(part 1 of 2)
# Autodesk Inventor assembly: 15InVEX
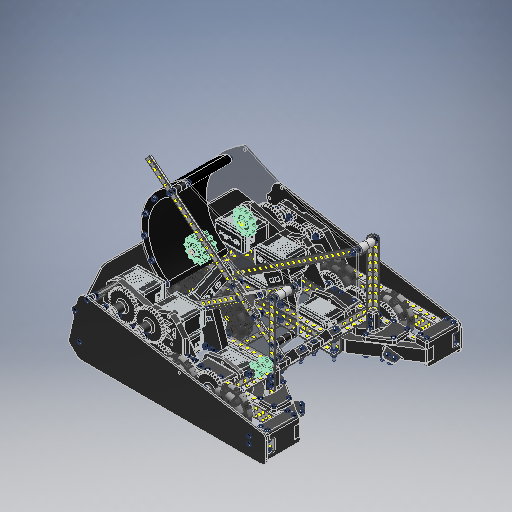
[picture p0: Inventor's stored thumbnail of the model, 512x512]
Saved by Autodesk Inventor 2026.1 (Build 301233000, 233)
## iProperties
Created: 2025-09-07
Part Number: 15InVEX
Document SubType Name: Assembly
Designer: Teddy
Mass: 633.16 g
Surface Area: 4744.79 cm^2
Volume: 520.993 cm^3
Density: 1.2153 g/cm^3
Author: Teddy
## Documents named in this file (80)
- C:\Users\Teddy\Desktop\VexCAD\15InVEX\15InVEX.iam
- C:\Users\Teddy\Desktop\VexCAD\VEX-CAD-Inventor\Structure\C Channel\Aluminum 1x2x1\Alu C 1x2x1x29.ipt
- C:\Users\Teddy\Desktop\VexCAD\VEX-CAD-Inventor\Structure\C Channel\Aluminum 1x3x1\Alu C 1x3x1x29.ipt
- C:\Users\Teddy\Desktop\VexCAD\VEX-CAD-Inventor\Motion\Wheels\Omni Wheel.iam
- C:\Users\Teddy\Desktop\VexCAD\VEX-CAD-Inventor\Structure\Hardware\Screw Steel - Star\SScrew Star Smooth 2.000.ipt
- C:\Users\Teddy\Desktop\VexCAD\VEX-CAD-Inventor\Structure\Hardware\Screw Steel - Star.ipt
- C:\Users\Teddy\Desktop\VexCAD\15InVEX\DriveGear1.ipt
- C:\Users\Teddy\Desktop\VexCAD\VEX-CAD-Inventor\Structure\Hardware\Nut Thin Nylock.ipt
- C:\Users\Teddy\Desktop\VexCAD\VEX-CAD-Inventor\Motion\Insert Circle.ipt
- C:\Users\Teddy\Desktop\VexCAD\15InVEX\DriveGear2.ipt
- C:\Users\Teddy\Desktop\VexCAD\VEX-CAD-Inventor\Motion\Spacers\Spacer Nylon .500 OD.ipt
- C:\Users\Teddy\Desktop\VexCAD\VEX-CAD-Inventor\Motion\Wheels\Omni Wheel\2.75 Omni AS, No Insert.iam
- C:\Users\Teddy\Desktop\VexCAD\VEX-CAD-Inventor\Motion\Insert Square.ipt
- C:\Users\Teddy\Desktop\VexCAD\VEX-CAD-Inventor\Motion\Spacers\Spacer Nylon .500 OD\NSpacer Black .500 OD x .125.ipt
- C:\Users\Teddy\Desktop\VexCAD\VEX-CAD-Inventor\Motion\Spacers\Washer Teflon\TWasher .375 OD x .06250.ipt
- C:\Users\Teddy\Desktop\VexCAD\VEX-CAD-Inventor\Motion\Spacers\Washer Teflon.ipt
- C:\Users\Teddy\Desktop\VexCAD\VEX-CAD-Inventor\Structure\Hardware\Screw Steel - Star\SScrew Star Smooth .250.ipt
- C:\Users\Teddy\Desktop\VexCAD\VEX-CAD-Inventor\Structure\Hardware\Nut Nylock.ipt
- C:\Users\Teddy\Desktop\VexCAD\VEX-CAD-Inventor\Motion\Spacers\Washer Teflon\TWasher .500 OD x .04000.ipt
- C:\Users\Teddy\Desktop\VexCAD\VEX-CAD-Inventor\Motion\Shaft LS\Bearing Flat.ipt
- C:\Users\Teddy\Desktop\VexCAD\VEX-CAD-Inventor\Structure\Hardware\Screw Steel - Star\SScrew Star Smooth .500.ipt
- C:\Users\Teddy\Desktop\VexCAD\VEX-CAD-Inventor\Motion\Spacers\Spacer Nylon .375 OD\NSpacer .375 OD x .250.ipt
- C:\Users\Teddy\Desktop\VexCAD\VEX-CAD-Inventor\Motion\Spacers\Spacer Nylon .375 OD.ipt
- C:\Users\Teddy\Desktop\VexCAD\VEX-CAD-Inventor\Motion\Spacers\Washer Teflon\TWasher .375 OD x .03125.ipt
- C:\Users\Teddy\Desktop\VexCAD\VEX-CAD-Inventor\Structure\Hardware\Screw Steel - Star\SScrew Star Smooth 1.000.ipt
- C:\Users\Teddy\Desktop\VexCAD\15InVEX\CapOriginal.ipt
- C:\Users\Teddy\Desktop\VexCAD\VEX-CAD-Inventor\Structure\Hardware\Screw Steel - Star\SScrew Star Smooth 1.500.ipt
- C:\Users\Teddy\Desktop\VexCAD\VEX-CAD-Inventor\Motion\Shaft LS\Shaft LS.ipt
- C:\Users\Teddy\Desktop\VexCAD\15InVEX\3rdAnd4thGearMount.ipt
- C:\Users\Teddy\Desktop\VexCAD\15InVEX\CombinedMotorMount.ipt
- C:\Users\Teddy\Desktop\VexCAD\VEX-CAD-Inventor\Structure\Hardware\Screw Steel - Star\SScrew Star Smooth .875.ipt
- C:\Users\Teddy\Desktop\VexCAD\VEX-CAD-Inventor\Structure\Hardware\Screw Steel - Star\SScrew Star Smooth 1.750.ipt
- C:\Users\Teddy\Desktop\VexCAD\VEX-CAD-Inventor\Motion\Shaft LS\Shaft LS\Shaft LS 3.5.ipt
- C:\Users\Teddy\Desktop\VexCAD\15InVEX\CombinedMotorMount_MIR.ipt
- C:\Users\Teddy\Desktop\VexCAD\15InVEX\3rdAnd4thGearMount_MIR.ipt
- C:\Users\Teddy\Desktop\VexCAD\15FEBOY\Clamp.ipt
- C:\Users\Teddy\Desktop\VexCAD\VEX-CAD-Inventor\Electronics\V5 Motor No Cap.ipt
- C:\Users\Teddy\Desktop\VexCAD\VEX-CAD-Inventor\Structure\Angle\Aluminum 1x1\Alu Angle 1x1x21.ipt
- C:\Users\Teddy\Desktop\VexCAD\VEX-CAD-Inventor\Structure\C Channel\Aluminum 1x2x1\Alu C 1x2x1x21.ipt
- C:\Users\Teddy\Desktop\VexCAD\VEX-CAD-Inventor\Motion\Spacers\Washer Steel\SWasher .375 OD x .031250.ipt
- C:\Users\Teddy\Desktop\VexCAD\VEX-CAD-Inventor\Motion\Spacers\Washer Steel.ipt
- C:\Users\Teddy\Desktop\VexCAD\VEX-CAD-Inventor\Structure\Hardware\Screw Steel - Star\SScrew Star Smooth .750.ipt
- C:\Users\Teddy\Desktop\VexCAD\15InVEX\Funnel.ipt
- C:\Users\Teddy\Desktop\VexCAD\15InVEX\HardStop.ipt
- C:\Users\Teddy\Desktop\VexCAD\15InVEX\Funnel_MIR.ipt
- C:\Users\Teddy\Desktop\VexCAD\15InVEX\PolyRamp1.ipt
- C:\Users\Teddy\Desktop\VexCAD\15InVEX\Ramp Support.ipt
- C:\Users\Teddy\Desktop\VexCAD\VEX-CAD-Inventor\Structure\Angle\Aluminum 1x1\Alu Angle 1x1x25.ipt
- C:\Users\Teddy\Desktop\VexCAD\15InVEX\AngleSupport.ipt
- C:\Users\Teddy\Desktop\VexCAD\VEX-CAD-Inventor\Structure\Hardware\Screw Steel - Star\SScrew Star Smooth .625.ipt
- C:\Users\Teddy\Desktop\VexCAD\15InVEX\AngleSupport_MIR.ipt
- C:\Users\Teddy\Desktop\VexCAD\VEX-CAD-Inventor\Structure\Angle\Aluminum 1x1\Alu Angle 1x1x15.ipt
- C:\Users\Teddy\Desktop\VexCAD\15InVEX\IntakeSupport.ipt
- C:\Users\Teddy\Desktop\VexCAD\VEX-CAD-Inventor\Motion\Spacers\Spacer Nylon .500 OD\NSpacer White .500 OD x .500.ipt
- C:\Users\Teddy\Desktop\VexCAD\VEX-CAD-Inventor\Motion\Spacers\Spacer Nylon .375 OD\NSpacer .375 OD x .500.ipt
- C:\Users\Teddy\Desktop\VexCAD\VEX-CAD-Inventor\Motion\Spacers\Spacer Nylon .375 OD\NSpacer .375 OD x .375.ipt
- C:\Users\Teddy\Desktop\VexCAD\VEX-CAD-Inventor\Structure\C Channel\Aluminum 1x2x1\Alu C 1x2x1x27.ipt
- C:\Users\Teddy\Desktop\VexCAD\15InVEX\IntakeSupport_MIR.ipt
- C:\Users\Teddy\Desktop\VexCAD\VEX-CAD-Inventor\Structure\Hardware\Screw Steel - Star\SScrew Star Smooth .375.ipt
- C:\Users\Teddy\Desktop\VexCAD\VEX-CAD-Inventor\Structure\Angle\Aluminum 1x1\Alu Angle 1x1x10.ipt
- C:\Users\Teddy\Desktop\VexCAD\VEX-CAD-Inventor\Motion\Wheels\Flex Wheels\1.625 Flex Wheel\1.625 30A .500.ipt
- C:\Users\Teddy\Desktop\VexCAD\VEX-CAD-Inventor\Motion\Wheels\Flex Wheels\1.625 Flex Wheel.ipt
- C:\Users\Teddy\Desktop\VexCAD\VEX-CAD-Inventor\Structure\Angle\Aluminum 1x1\Alu Angle 1x1x26.ipt
- C:\Users\Teddy\Desktop\VexCAD\15InVEX\TwistySupport.ipt
- C:\Users\Teddy\Desktop\VexCAD\VEX-CAD-Inventor\Motion\Sprockets\9P Sprocket\9P 6T Sprocket, Circle.iam
- C:\Users\Teddy\Desktop\VexCAD\VEX-CAD-Inventor\Motion\Sprockets\9P Sprocket.iam
- C:\Users\Teddy\Desktop\VexCAD\VEX-CAD-Inventor\Motion\Spacers\Spacer Nylon .375 OD\NSpacer .375 OD x .125.ipt
- C:\Users\Teddy\Desktop\VexCAD\VEX-CAD-Inventor\Structure\Hardware\Screw Steel - Star\SScrew Star Smooth 2.500.ipt
- C:\Users\Teddy\Desktop\VexCAD\15InVEX\PolyIntakeSides.ipt
- C:\Users\Teddy\Desktop\VexCAD\VEX-CAD-Inventor\Structure\Standoff\Standoff 4.00.ipt
- C:\Users\Teddy\Desktop\VexCAD\VEX-CAD-Inventor\Structure\Standoff.ipt
- C:\Users\Teddy\Desktop\VexCAD\VEX-CAD-Inventor\Motion\Sprockets\9P Sprocket\9P 12T Sprocket, No Insert.iam
- C:\Users\Teddy\Desktop\VexCAD\VEX-CAD-Inventor\Motion\Shaft HS\HS Spacer\HSpacer .1250.ipt
- C:\Users\Teddy\Desktop\VexCAD\VEX-CAD-Inventor\Motion\Shaft HS\HS Spacer.ipt
- C:\Users\Teddy\Desktop\VexCAD\15InVEX\ChassisPolySides.ipt
- C:\Users\Teddy\Desktop\VexCAD\VEX-CAD-Inventor\Structure\Standoff\Standoff 1.50.ipt
- C:\Users\Teddy\Desktop\VexCAD\VEX-CAD-Inventor\Structure\Standoff\Standoff .50.ipt
- C:\Users\Teddy\Desktop\VexCAD\15InVEX\Mesh.ipt
- C:\Users\Teddy\Desktop\VexCAD\15InVEX\BackPoly.ipt
- C:\Users\Teddy\Desktop\VexCAD\VEX-CAD-Inventor\Electronics\Sensors\V5 Rotation Sensor.ipt
## Components (575 placed, 68 different names)
1. SScrew Star Smooth .375:135 — Insert:576
2. SScrew Star Smooth .375:136 — Insert:577
3. Nut Nylock:188 — Insert:579
4. Nut Nylock:189 — Insert:578
5. Alu Angle 1x1x10:1 — Insert:580, Insert:581, Insert:604
6. 1.625 30A .500:1 — Insert:581
7. 1.625 30A .500:2
8. Alu Angle 1x1x26:1 — Insert:582, Flush:20, Insert:584, Insert:585, Insert:586, Insert:587, Insert:598, Insert:599, Insert:606, Insert:607
9. TwistySupport:1 — Flush:18, Flush:19, Flush:20, Insert:583, Insert:584, Insert:585, Insert:588, Insert:589, Insert:590, Insert:593
10. SScrew Star Smooth .750:137 — Insert:586
11. SScrew Star Smooth .750:138 — Insert:587
12. SScrew Star Smooth .750:139 — Insert:588
13. SScrew Star Smooth .750:140 — Insert:589
14. Nut Nylock:190 — Insert:593
15. Nut Nylock:191 — Insert:592
16. Nut Nylock:192 — Insert:591
17. Nut Nylock:193 — Insert:590
18. 9P 6T Sprocket, Circle:1 [sub-assembly] — Insert:595, Insert:597
19. 9P 6T Sprocket, Circle:2 [sub-assembly] — Insert:594, Insert:603
20. NSpacer .375 OD x .125:13 — Insert:594, Insert:597
21. NSpacer .375 OD x .125:15 — Insert:595, Insert:580
22. SScrew Star Smooth 2.500:141 — Insert:598
23. Nut Nylock:194 — Insert:599
24. Nut Nylock:195 — Insert:601, Insert:603
25. Nut Nylock:196 — Insert:600, Insert:602
26. TWasher .500 OD x .04000:21 — Insert:602
27. Nut Nylock:197 — Insert:605
28. TWasher .500 OD x .04000:22 — Insert:604, Insert:605
29. PolyIntakeSides:1 — Flush:21, Flush:22, Insert:560, Insert:592, Insert:591, Insert:610, Insert:618, Insert:620, Insert:621, Insert:622, Insert:623, Insert:624, Insert:625, Insert:626, Insert:645, Insert:657, Insert:658, Insert:659, Insert:660, Insert:661, Insert:662
30. SScrew Star Smooth 1.500:142 — Insert:606
31. Nut Nylock:198 — Insert:607, Insert:608
32. Nut Nylock:199 — Insert:610
33. NSpacer .375 OD x .375:16 — Insert:608, Insert:609
34. NSpacer .375 OD x .375:17 — Insert:609
35. SScrew Star Smooth 2.000:143 — Insert:611
36. Nut Nylock:200 — Insert:612, Insert:613
37. NSpacer .375 OD x .500:18 — Insert:614, Insert:615
38. NSpacer .375 OD x .500:20 — Insert:613, Insert:614
39. NSpacer .375 OD x .250:22 — Insert:615, Insert:616
40. TWasher .500 OD x .04000:23 — Insert:616, Insert:617
41. TWasher .500 OD x .04000:24 — Insert:617
42. Nut Nylock:201 — Insert:618
43. SScrew Star Smooth .375:144 — Insert:619
44. Nut Nylock:202 — Insert:620
45. Standoff 4.00:1 — Insert:631, Insert:638
46. Standoff 4.00:2 — Insert:630, Insert:636
47. Standoff 4.00:3 — Insert:629, Insert:635
48. Standoff 4.00:4 — Insert:628, Insert:634
49. Standoff 4.00:5 — Insert:627, Insert:633
50. Standoff 4.00:6 — Insert:632, Insert:637
51. Nut Thin Nylock:24 — Insert:621, Insert:632
52. Nut Thin Nylock:25 — Insert:622, Insert:631
53. Nut Thin Nylock:26 — Insert:623, Insert:630
54. Nut Thin Nylock:27 — Insert:624, Insert:629
55. Nut Thin Nylock:28 — Insert:625, Insert:628
56. Nut Thin Nylock:29 — Insert:626, Insert:627
57. Nut Thin Nylock:30 — Insert:635, Insert:642
58. Nut Thin Nylock:31 — Insert:636, Insert:641
59. Nut Thin Nylock:32 — Insert:638, Insert:640
60. Nut Thin Nylock:33 — Insert:637, Insert:639
61. Nut Thin Nylock:34 — Insert:633, Insert:644
62. Nut Thin Nylock:35 — Insert:634, Insert:643
63. PolyIntakeSides:2 — Insert:639, Insert:640, Insert:641, Insert:642, Insert:643, Insert:644, Insert:646, Insert:651, Insert:652, Insert:653, Insert:654, Insert:655, Insert:656, Flush:26, Flush:27
64. 9P 12T Sprocket, No Insert:3 [sub-assembly] — Insert:650
65. 9P 12T Sprocket, No Insert:4 [sub-assembly] — Insert:648, Insert:649
66. 9P 12T Sprocket, No Insert:5 [sub-assembly] — Insert:647
67. HSpacer .1250:1 — Insert:645, Insert:648
68. HSpacer .1250:2 — Insert:649, Insert:650
69. HSpacer .1250:3 — Insert:646, Insert:647
70. SScrew Star Smooth .750:145 — Insert:651
71. SScrew Star Smooth .750:146 — Insert:652
72. SScrew Star Smooth .750:147 — Insert:654
73. SScrew Star Smooth .750:148 — Insert:653
74. SScrew Star Smooth .750:149 — Insert:655
75. SScrew Star Smooth .750:150 — Insert:656
76. SScrew Star Smooth .750:151 — Insert:658
77. SScrew Star Smooth .750:152 — Insert:657
78. SScrew Star Smooth .750:153 — Insert:659
79. SScrew Star Smooth .750:154 — Insert:662
80. SScrew Star Smooth .750:155 — Insert:661
81. SScrew Star Smooth .750:156 — Insert:660
82. ChassisPolySides:1 — Flush:24, Flush:25, Insert:665, Insert:666, Insert:669, Insert:670, Insert:673, Insert:674, Insert:675, Insert:676, Insert:677, Insert:678
83. Standoff 1.50:7 — Insert:663, Insert:667
84. Standoff 1.50:8 — Insert:664, Insert:668
85. SScrew Star Smooth 1.000:157 — Insert:665
86. SScrew Star Smooth 1.000:158 — Insert:666
87. Nut Nylock:203 — Insert:667
88. Nut Nylock:204 — Insert:668
89. Nut Nylock:205 — Insert:670, Insert:672
90. Nut Nylock:206 — Insert:669, Insert:671
91. NSpacer .375 OD x .125:23 — Insert:671
92. NSpacer .375 OD x .125:24 — Insert:672
93. SScrew Star Smooth 1.000:159 — Insert:674
94. SScrew Star Smooth 1.000:160 — Insert:675
95. SScrew Star Smooth 1.000:161 — Insert:673
96. Standoff .50:9 — Insert:677
97. Standoff .50:10 — Insert:676
98. Standoff .50:11 — Insert:678
99. Nut Nylock:207 — Insert:679
100. Nut Nylock:208 — Insert:681
101. Nut Nylock:209 — Insert:680
102. ChassisPolySides:2 — Insert:682, Insert:683, Insert:684
103. Mesh:1 — Flush:26, Flush:27
104. BackPoly:1 — Flush:28, Flush:29, Insert:685, Insert:686, Insert:687, Insert:688
105. SScrew Star Smooth .500:162 — Insert:685
106. SScrew Star Smooth .500:163 — Insert:686
107. SScrew Star Smooth .500:164 — Insert:687
108. SScrew Star Smooth .500:165 — Insert:688
109. 2.75 Omni AS, No Insert:7 [sub-assembly] — Insert:689, Insert:691
110. 2.75 Omni AS, No Insert:8 [sub-assembly] — Insert:690, Insert:692
111. V5 Rotation Sensor:1 — Insert:691
112. V5 Rotation Sensor:2 — Insert:692
113. Alu Angle 1x1x15:2 — Insert:556, Insert:557, Insert:559, Insert:570, Insert:571, Angle:13, Insert:582, Insert:600, Insert:601, Insert:611, Insert:612
114. Alu Angle 1x1x15:1 — Insert:507, Angle:12, Insert:514, Insert:515, Insert:535, Insert:536
115. Alu Angle 1x1x25:2 — Insert:491, Insert:495, Insert:496, Insert:497, Insert:498, Insert:556, Insert:558, Flush:18, Flush:19, Insert:583, Flush:21, Flush:22, Insert:619
116. Alu Angle 1x1x25:1 — Insert:476, Insert:479, Insert:480, Insert:489, Insert:490, Insert:507, Insert:516, Insert:517
117. Alu C 1x2x1x21:2 — Insert:344, Insert:345, Insert:351, Insert:353, Insert:354, Insert:359, Insert:360, Insert:364, Insert:367, Insert:368, Insert:375, Insert:491, Insert:492, Insert:493, Insert:494, Insert:504, Insert:505, Insert:506, Insert:576, Insert:577, Flush:23, Insert:689
118. Alu C 1x2x1x21:1 — Insert:343, Insert:346, Insert:352, Insert:355, Insert:356, Insert:361, Insert:362, Insert:363, Insert:372, Insert:373, Insert:376, Insert:476, Flush:13, Mate:19, Mate:20, Insert:481, Insert:482, Insert:483, Insert:484, Insert:485
119. Alu C 1x3x1x29:1 — Insert:1, Angle:1, Insert:29, Insert:141, Insert:144, Insert:155, Insert:305, Insert:306, Angle:5, Insert:345, Insert:346, Insert:365, Insert:366, Insert:369, Insert:370, Insert:371, Insert:374, Flush:28, Flush:29, Insert:690
120. Alu Angle 1x1x21:2 — Insert:333, Insert:334, Insert:165, Insert:296, Insert:357, Insert:358
121. Alu Angle 1x1x21:1 — Insert:331, Insert:332, Insert:335, Insert:336, Insert:343, Insert:344, Mate:14, Insert:421, Insert:422, Insert:436, Insert:466, Insert:470
122. V5 Motor No Cap:7 — Mate:17, Insert:474, Angle:10
123. V5 Motor No Cap:8 — Mate:18, Insert:475, Angle:11
124. V5 Motor No Cap:5 — Mate:12, Insert:348, Angle:9
125. V5 Motor No Cap:6 — Mate:11, Insert:347, Angle:8
126. V5 Motor No Cap:3 — Mate:9, Insert:327
127. V5 Motor No Cap:4 — Mate:10, Insert:328
128. V5 Motor No Cap:1 — Mate:7, Insert:325
129. V5 Motor No Cap:2 — Mate:8, Insert:326
130. Nut Nylock:186 — Insert:570
131. Nut Nylock:187 — Insert:571
132. Nut Nylock:183 — Insert:558
133. Nut Nylock:184 — Insert:559, Insert:561
134. Nut Nylock:185 — Insert:560
135. Nut Nylock:181 — Insert:535
136. Nut Nylock:182 — Insert:536
137. Nut Nylock:177 — Insert:525
138. Nut Nylock:178 — Insert:526
139. Nut Nylock:179 — Insert:527
140. Nut Nylock:180 — Insert:528
141. Nut Nylock:174 — Insert:517, Insert:518
142. Nut Nylock:175 — Insert:516
143. Nut Nylock:176 — Insert:515
144. Nut Nylock:169 — Insert:501
145. Nut Nylock:170 — Insert:502
146. Nut Nylock:171 — Insert:503
147. Nut Nylock:172 — Insert:499
148. Nut Nylock:173 — Insert:500
149. Nut Nylock:164 — Insert:477
150. Nut Nylock:165 — Insert:478
151. Nut Nylock:166 — Insert:486
152. Nut Nylock:167 — Insert:488
153. Nut Nylock:168 — Insert:487
154. Nut Nylock:161 — Insert:460
155. Nut Nylock:162 — Insert:470
156. Nut Nylock:163 — Insert:471
157. Nut Nylock:143 — Insert:436
158. Nut Nylock:142 — Insert:430
159. Nut Nylock:137 — Insert:417
160. Nut Nylock:138 — Insert:419
161. Nut Nylock:139 — Insert:418
162. Nut Nylock:140 — Insert:420
163. Nut Nylock:115 — Insert:367
164. Nut Nylock:116 — Insert:368
165. Nut Nylock:117 — Insert:369
166. Nut Nylock:118 — Insert:372
167. Nut Nylock:119 — Insert:370
168. Nut Nylock:120 — Insert:371
169. Nut Nylock:121 — Insert:373
170. Nut Nylock:122 — Insert:374
171. Nut Nylock:109 — Insert:361
172. Nut Nylock:110 — Insert:360
173. Nut Nylock:111 — Insert:363
174. Nut Nylock:112 — Insert:362
175. Nut Nylock:113 — Insert:364
176. Nut Nylock:114 — Insert:359
177. Nut Nylock:103 — Insert:351
178. Nut Nylock:104 — Insert:352
179. Nut Nylock:105 — Insert:355
180. Nut Nylock:106 — Insert:353
181. Nut Nylock:107 — Insert:354
182. Nut Nylock:108 — Insert:356
183. SScrew Star Smooth 1.500:129 — Insert:564
184. SScrew Star Smooth 1.500:130 — Insert:565
185. SScrew Star Smooth 1.500:131 — Insert:566
186. SScrew Star Smooth 1.500:132 — Insert:567
187. SScrew Star Smooth .750:133 — Insert:568
188. SScrew Star Smooth .750:134 — Insert:569
189. SScrew Star Smooth 2.000:128 — Insert:557
190. SScrew Star Smooth .750:126 — Insert:540
191. SScrew Star Smooth .750:127 — Insert:541
192. SScrew Star Smooth 1.500:122 — Insert:539
193. SScrew Star Smooth 1.500:123
194. SScrew Star Smooth 1.500:124 — Insert:538
195. SScrew Star Smooth 1.500:125
196. SScrew Star Smooth 2.000:121 — Insert:514
197. SScrew Star Smooth .750:118 — Insert:504
198. SScrew Star Smooth .750:119 — Insert:505
199. SScrew Star Smooth .750:120 — Insert:506
200. SScrew Star Smooth .750:111 — Insert:484
201. SScrew Star Smooth .750:112 — Insert:483
202. SScrew Star Smooth .750:113 — Insert:485
203. SScrew Star Smooth .625:114 — Insert:489
204. SScrew Star Smooth .625:115 — Insert:490
205. SScrew Star Smooth 1.750:108 — Insert:467
206. SScrew Star Smooth .875:109 — Insert:468
207. SScrew Star Smooth .875:110 — Insert:469
208. SScrew Star Smooth .750:86 — Insert:428
209. SScrew Star Smooth .750:87 — Insert:429
210. SScrew Star Smooth 2.000:88 — Insert:432
211. SScrew Star Smooth .750:82 — Insert:423
212. SScrew Star Smooth .750:83 — Insert:414
213. SScrew Star Smooth .750:84 — Insert:424
214. SScrew Star Smooth .750:85 — Insert:425
215. SScrew Star Smooth 1.500:72 — Insert:358
216. SScrew Star Smooth 1.500:73 — Insert:357
217. SScrew Star Smooth 2.000:74 — Insert:366
218. SScrew Star Smooth 2.000:75 — Insert:365
219. NSpacer .375 OD x .500:9 — Insert:572, Insert:574
220. NSpacer .375 OD x .500:10 — Insert:573, Insert:575
221. NSpacer .375 OD x .375:11 — Insert:574
222. NSpacer .375 OD x .375:12 — Insert:575
223. NSpacer White .500 OD x .500:18 — Insert:561, Insert:562
224. NSpacer White .500 OD x .500:19 — Insert:562, Insert:563
225. TWasher .500 OD x .04000:20 — Insert:563
226. NSpacer .375 OD x .500:5 — Insert:529, Insert:532
227. NSpacer .375 OD x .500:6 — Insert:530, Insert:531
228. NSpacer .375 OD x .375:7 — Insert:531
229. NSpacer .375 OD x .375:8 — Insert:532
230. NSpacer White .500 OD x .500:16 — Insert:518, Insert:519
231. NSpacer White .500 OD x .500:17 — Insert:519, Insert:520
232. TWasher .500 OD x .04000:19 — Insert:520
233. SScrew Star Smooth .625:116 — Insert:497
234. SScrew Star Smooth .625:117 — Insert:498
235. NSpacer Black .500 OD x .125:14 — Insert:376, Insert:378
236. NSpacer Black .500 OD x .125:15 — Insert:375, Insert:377
237. SWasher .375 OD x .031250:1 — Insert:377
238. SWasher .375 OD x .031250:2 — Insert:378
239. IntakeSupport_MIR:1 — Insert:552, Insert:553, Insert:554, Insert:555, Insert:564, Insert:565, Insert:566, Insert:567, Insert:568, Insert:569
240. HardStop:3 — Insert:542, Insert:543, Insert:544, Insert:545, Insert:546, Insert:547
241. AngleSupport_MIR:1 — Insert:492, Insert:493, Insert:494, Insert:495, Insert:496, Insert:499, Insert:500, Insert:501, Insert:502, Insert:503
242. IntakeSupport:1 — Flush:14, Flush:15, Flush:16, Insert:509, Insert:510, Insert:538, Insert:539, Insert:540, Insert:541
243. AngleSupport:1 — Flush:13, Mate:19, Mate:20, Insert:477, Insert:478, Insert:479, Insert:480, Insert:481, Insert:482, Insert:486, Insert:487, Insert:488
244. Funnel:1 — Mate:13, Mate:14, Mate:16, Insert:419, Insert:420, Insert:413, Insert:543, Insert:552, Insert:553, Insert:578, Insert:579
245. Funnel_MIR:1 — Insert:417, Insert:418, Flush:14, Flush:15, Insert:525, Insert:526, Insert:537
246. Ramp Support:1 — Insert:421, Insert:430, Insert:432, Insert:469
247. Ramp Support:2 — Insert:422, Insert:466, Insert:467, Insert:468, Insert:471
248. PolyRamp1:1 — Insert:413, Insert:414, Insert:423, Insert:424, Insert:425, Insert:428, Insert:429
249. Alu C 1x2x1x27:2 — Insert:1, Insert:10, Insert:11, Angle:1, Insert:17, Insert:24, Insert:45, Insert:59, Insert:63, Insert:64, Insert:87, Mate:1, Angle:2, Insert:91, Insert:92, Insert:93, Insert:94, Insert:95, Insert:96, Insert:101, Insert:102, Insert:109, Insert:110, Insert:111, Insert:112, Insert:113, Insert:114, Insert:123, Insert:124, Insert:156, Insert:157, Insert:160, Insert:161, Insert:162, Insert:163, Insert:164, Angle:4, Insert:331, Insert:334, Insert:340, Insert:341, Insert:342, Mate:13, Insert:554, Insert:555, Insert:572, Insert:573
250. Alu C 1x2x1x29:3 — Insert:29, Insert:32, Insert:33, Insert:34, Insert:35, Insert:36, Insert:48, Insert:49, Insert:85, Insert:86, Flush:2, Flush:3, Flush:4, Insert:145, Insert:146, Insert:147, Insert:148, Insert:149, Insert:150, Insert:151, Insert:152, Insert:168, Insert:169, Mate:16, Insert:456, Insert:457, Insert:458, Insert:459, Insert:460, Insert:461, Insert:473, Insert:542, Angle:13, Flush:24, Flush:25, Insert:679, Insert:680, Insert:681
251. Clamp:4 — Insert:323
252. Clamp:1 — Insert:324
253. CapOriginal:1 — Insert:87, Mate:1, Angle:2, Insert:88, Insert:89, Insert:90, Insert:97, Insert:98, Insert:99, Insert:323, Mate:7, Insert:325
254. CapOriginal:2 — Insert:101, Insert:102, Insert:103, Insert:104, Insert:105, Insert:106, Insert:107, Insert:108, Insert:324, Mate:8, Insert:326
255. CombinedMotorMount:1 — Insert:123, Insert:124, Insert:158, Insert:159, Mate:12, Insert:348, Angle:9, Mate:17, Insert:474, Angle:10, Insert:663, Insert:664
256. 3rdAnd4thGearMount:1 — Flush:2, Flush:3, Flush:4, Insert:119, Insert:127, Insert:128, Insert:129, Insert:130, Insert:137, Insert:138, Insert:139, Insert:140, Insert:170, Insert:171, Insert:472, Insert:473
257. DriveGear1:1 — Insert:12, Insert:20, Insert:57, Insert:58, Rotation:4
258. DriveGear1:2 — Insert:18, Insert:50, Insert:51, Insert:52, Insert:54, Insert:55, Insert:56, Rotation:2, Rotation:3
259. DriveGear2:1 — Insert:21, Insert:25, Insert:39, Tangent:1, Flush:1, Rotation:3, Rotation:4, Rotation:5
260. DriveGear2:2 — Insert:46, Insert:78, Insert:81, Rotation:1, Rotation:2
261. DriveGear1:3 — Insert:65, Insert:66, Insert:67, Insert:69, Insert:70, Insert:71, Rotation:1
262. DriveGear2:3 — Tangent:1, Flush:1, Insert:115, Tangent:2, Flush:6, Insert:125, Insert:154, Rotation:5, Rotation:6
263. DriveGear2:4 — Tangent:2, Flush:6, Insert:119, Insert:120, Insert:126, Insert:153, Rotation:6
264. 2.75 Omni AS, No Insert:1 [sub-assembly] — Insert:20, Insert:26, Insert:72, Insert:73
265. 2.75 Omni AS, No Insert:2 [sub-assembly] — Insert:50, Insert:51, Insert:52, Insert:54, Insert:60, Insert:74, Insert:75
266. 2.75 Omni AS, No Insert:3 [sub-assembly] — Insert:69, Insert:70, Insert:71, Insert:76, Insert:77, Insert:82
267. NSpacer Black .500 OD x .125:1 — Insert:22, Insert:23
268. TWasher .375 OD x .06250:1 — Insert:23, Insert:24
269. TWasher .500 OD x .04000:2 — Insert:31
270. NSpacer .375 OD x .250:1 — Insert:40, Insert:41
271. TWasher .375 OD x .03125:3 — Insert:41
272. TWasher .375 OD x .06250:4 — Insert:44, Insert:45
273. NSpacer Black .500 OD x .125:2 — Insert:44, Insert:47
274. TWasher .500 OD x .04000:5 — Insert:62
275. NSpacer .375 OD x .250:2 — Insert:79, Insert:80
276. TWasher .375 OD x .03125:6 — Insert:80
277. TWasher .500 OD x .04000:7 — Insert:84
278. NSpacer Black .500 OD x .125:3 — Insert:116, Insert:117
279. TWasher .375 OD x .06250:8 — Insert:117
280. NSpacer Black .500 OD x .125:4 — Insert:121, Insert:122
281. TWasher .375 OD x .06250:9 — Insert:122
282. NSpacer Black .500 OD x .125:6 — Insert:131
283. NSpacer Black .500 OD x .125:7 — Insert:132
284. Insert Circle:1 — Insert:12, Insert:13
285. Insert Circle:3 — Insert:18, Insert:19
286. Insert Square:1 — Insert:21, Insert:22
287. Insert Circle:4 — Insert:26, Insert:30
288. Insert Square:2 — Insert:39, Insert:40
289. Insert Square:3 — Insert:46, Insert:47
290. Insert Circle:5 — Insert:60, Insert:61
291. Insert Circle:6 — Insert:65, Insert:68
292. Insert Square:4 — Insert:78, Insert:79
293. Insert Circle:7 — Insert:82, Insert:83
294. Insert Square:5 — Insert:115, Insert:116
295. Insert Square:6 — Insert:120, Insert:121
296. Insert Square:7 — Insert:125, Insert:131
297. Insert Square:8 — Insert:126, Insert:132
298. Bearing Flat:1 — Insert:33, Insert:34, Insert:37, Insert:38, Insert:172
299. Bearing Flat:2 — Insert:48, Insert:49, Insert:166, Insert:167, Insert:330
300. Bearing Flat:3 — Insert:127, Insert:128, Insert:135, Insert:136
301. Bearing Flat:4 — Insert:129, Insert:130, Insert:133, Insert:134
302. Nut Nylock:154 — Insert:457
303. Nut Nylock:155 — Insert:459
304. Nut Nylock:156 — Insert:458
305. Nut Nylock:157 — Insert:456
306. Nut Nylock:158
307. Nut Nylock:159 — Insert:461
308. Nut Nylock:160
309. Nut Nylock:100 — Insert:342
310. Nut Nylock:101 — Insert:341
311. Nut Nylock:102 — Insert:340
312. Nut Thin Nylock:1 — Insert:11, Insert:13
313. Nut Thin Nylock:3 — Insert:17, Insert:19
314. Nut Thin Nylock:4 — Insert:37
315. Nut Thin Nylock:5 — Insert:38
316. Nut Nylock:1 — Insert:30, Insert:31
317. Nut Nylock:2 — Insert:32
318. Nut Nylock:3 — Insert:61, Insert:62
319. Nut Thin Nylock:6 — Insert:64, Insert:68
320. Nut Thin Nylock:7 — Insert:72
321. Nut Thin Nylock:8 — Insert:73
322. Nut Thin Nylock:9 — Insert:74
323. Nut Thin Nylock:10 — Insert:75
324. Nut Thin Nylock:11 — Insert:76
325. Nut Thin Nylock:12 — Insert:77
326. Nut Nylock:4 — Insert:83, Insert:84
327. Nut Nylock:5 — Insert:86
328. Nut Nylock:6 — Insert:85
329. Nut Nylock:7 — Insert:93
330. Nut Nylock:8 — Insert:91
331. Nut Nylock:9 — Insert:92
332. Nut Nylock:10 — Insert:97
333. Nut Nylock:11 — Insert:94
334. Nut Nylock:12 — Insert:95
335. Nut Nylock:13 — Insert:98
336. Nut Nylock:14 — Insert:99
337. Nut Nylock:15 — Insert:96
338. Nut Nylock:16 — Insert:106
339. Nut Nylock:17 — Insert:107
340. Nut Nylock:18 — Insert:108
341. Nut Nylock:19 — Insert:109
342. Nut Nylock:20 — Insert:110
343. Nut Nylock:21 — Insert:111
344. Nut Nylock:22 — Insert:112
345. Nut Nylock:23 — Insert:113
346. Nut Nylock:24 — Insert:114
347. Nut Nylock:25
348. Nut Nylock:26 — Insert:133
349. Nut Nylock:27 — Insert:134
350. Nut Nylock:28 — Insert:135
351. Nut Nylock:29 — Insert:136
352. Nut Nylock:30 — Insert:141
353. Nut Nylock:31
354. Nut Nylock:32 — Insert:472
355. Nut Nylock:33 — Insert:149
356. Nut Nylock:34 — Insert:150
357. Nut Nylock:35 — Insert:151
358. Nut Nylock:36 — Insert:147
359. Nut Nylock:37 — Insert:148
360. Nut Nylock:38 — Insert:152
361. Nut Nylock:39 — Insert:156
362. Nut Nylock:40 — Insert:157
363. Nut Nylock:41 — Insert:160
364. Nut Nylock:42 — Insert:161
365. Nut Nylock:43 — Insert:162
366. Nut Nylock:44 — Insert:163
367. Nut Nylock:45 — Insert:165
368. Nut Nylock:46 — Insert:164
369. Nut Nylock:47 — Insert:166
370. Nut Nylock:48 — Insert:167
371. SScrew Star Smooth 1.750:104 — Insert:547
372. SScrew Star Smooth 1.750:105 — Insert:545
373. SScrew Star Smooth 1.750:106 — Insert:546
374. SScrew Star Smooth 1.750:107 — Insert:544
375. SScrew Star Smooth 1.500:68 — Insert:335
376. SScrew Star Smooth 2.000:1 — Insert:10
377. SScrew Star Smooth .250:2 — Insert:25
378. SScrew Star Smooth .500:3 — Insert:36
379. SScrew Star Smooth .500:4 — Insert:35
380. SScrew Star Smooth 1.000:5 — Insert:55
381. SScrew Star Smooth 1.000:6 — Insert:56
382. SScrew Star Smooth 1.000:7 — Insert:58
383. SScrew Star Smooth 1.000:8 — Insert:57
384. SScrew Star Smooth 2.000:9 — Insert:59
385. SScrew Star Smooth 1.000:12 — Insert:67
386. SScrew Star Smooth 2.000:10 — Insert:63
387. SScrew Star Smooth 1.000:13 — Insert:66
388. SScrew Star Smooth .250:14 — Insert:81
389. SScrew Star Smooth 1.500:15 — Insert:88
390. SScrew Star Smooth 1.500:16 — Insert:89
391. SScrew Star Smooth 1.500:17 — Insert:90
392. SScrew Star Smooth 1.500:18 — Insert:103
393. SScrew Star Smooth 1.500:19 — Insert:104
394. SScrew Star Smooth 1.500:20 — Insert:105
395. SScrew Star Smooth .875:21 — Insert:137
396. SScrew Star Smooth .875:22 — Insert:138
397. SScrew Star Smooth .875:23 — Insert:139
398. SScrew Star Smooth .875:24 — Insert:140
399. SScrew Star Smooth 1.750:25 — Insert:144
400. SScrew Star Smooth 1.750:26 — Insert:145
401. SScrew Star Smooth 1.500:27 — Insert:146
402. SScrew Star Smooth .250:28 — Insert:153
403. SScrew Star Smooth .250:29 — Insert:154
404. SScrew Star Smooth 1.750:30 — Insert:155
405. SScrew Star Smooth 1.500:31 — Insert:158
406. SScrew Star Smooth 1.500:32 — Insert:159
407. SScrew Star Smooth .500:33 — Insert:168
408. SScrew Star Smooth .500:34 — Insert:169
409. Shaft LS 3.5:9 — Insert:330
410. Shaft LS 3.5:2 — Insert:170
411. Shaft LS 3.5:3 — Insert:172
412. Shaft LS 3.5:4 — Insert:171
413. Alu C 1x2x1x27:1 — Insert:173, Insert:174, Insert:175, Insert:177, Insert:194, Insert:204, Insert:208, Insert:209, Insert:229, Angle:3, Insert:233, Insert:234, Insert:235, Insert:237, Insert:238, Insert:241, Insert:243, Insert:244, Insert:251, Insert:252, Insert:253, Insert:254, Insert:255, Insert:256, Insert:260, Insert:261, Insert:288, Insert:289, Insert:292, Insert:293, Insert:294, Insert:295, Insert:297, Insert:305, Angle:4, Insert:308, Insert:332, Insert:333, Insert:337, Insert:338, Insert:339, Flush:16, Insert:509, Insert:510, Insert:527, Insert:528, Insert:529, Insert:530
414. Alu C 1x2x1x29:5 — Insert:182, Insert:185, Insert:186, Insert:187, Insert:188, Insert:189, Insert:190, Insert:227, Insert:228, Mate:4, Mate:5, Mate:6, Insert:280, Insert:281, Insert:282, Insert:283, Insert:284, Insert:285, Insert:286, Insert:287, Insert:300, Insert:301, Insert:306, Angle:5, Insert:307, Insert:442, Insert:443, Insert:444, Insert:445, Insert:446, Insert:447, Angle:12, Insert:682, Insert:683, Insert:684
415. HardStop:2 — Insert:537, Insert:548, Insert:549, Insert:550, Insert:551
416. Clamp:2 — Insert:321, Angle:6
417. Clamp:3 — Insert:322, Angle:7
418. DriveGear1:4 — Insert:176, Insert:202, Insert:203
419. DriveGear1:5 — Insert:196, Insert:197, Insert:198, Insert:199, Insert:200, Insert:201
420. DriveGear2:5 — Insert:191, Flush:7, Tangent:3, Insert:310, Insert:319
421. CapOriginal:3 — Insert:229, Angle:3, Insert:230, Insert:231, Insert:232, Insert:236, Insert:239, Insert:240, Insert:308, Insert:321, Angle:6, Mate:9, Insert:327
422. CapOriginal:4 — Insert:243, Insert:244, Insert:245, Insert:246, Insert:247, Insert:248, Insert:249, Insert:250, Insert:322, Mate:10, Insert:328
423. CombinedMotorMount_MIR:1 — Insert:260, Insert:261, Insert:290, Insert:291, Angle:7, Mate:11, Insert:347, Angle:8, Mate:18, Insert:475, Angle:11
424. 3rdAnd4thGearMount_MIR:1 — Mate:4, Mate:5, Mate:6, Insert:265, Insert:266, Insert:267, Insert:268, Insert:274, Insert:275, Insert:276, Insert:277, Insert:302, Insert:304, Insert:307
425. DriveGear2:6 — Insert:221, Insert:309, Insert:320
426. DriveGear1:6 — Insert:210, Insert:211, Insert:212, Insert:213, Insert:214
427. DriveGear2:7 — Flush:7, Tangent:3, Flush:8, Tangent:4, Insert:262, Insert:311, Insert:318
428. DriveGear2:8 — Flush:8, Tangent:4, Insert:263, Insert:315, Insert:317
429. 2.75 Omni AS, No Insert:6 [sub-assembly] — Insert:212, Insert:213, Insert:214, Insert:219, Insert:220, Insert:224
430. 2.75 Omni AS, No Insert:4 [sub-assembly] — Insert:176, Insert:179, Insert:215, Insert:216
431. 2.75 Omni AS, No Insert:5 [sub-assembly] — Insert:196, Insert:197, Insert:198, Insert:199, Insert:205, Insert:217, Insert:218
432. Bearing Flat:5 — Insert:183, Insert:184, Insert:185, Insert:186, Insert:303
433. Bearing Flat:6 — Insert:187, Insert:188, Insert:298, Insert:299, Insert:329
434. Bearing Flat:7 — Insert:265, Insert:266, Insert:272, Insert:273, Insert:314
435. Bearing Flat:8 — Insert:267, Insert:268, Insert:270, Insert:271
436. NSpacer Black .500 OD x .125:8 — Insert:178, Insert:313
437. TWasher .375 OD x .06250:10 — Insert:177, Insert:178
438. TWasher .500 OD x .04000:11 — Insert:181
439. NSpacer .375 OD x .250:3 — Insert:192, Insert:193
440. TWasher .375 OD x .03125:12 — Insert:193
441. TWasher .375 OD x .06250:13 — Insert:194, Insert:195
442. NSpacer Black .500 OD x .125:9 — Insert:195, Insert:312
443. TWasher .500 OD x .04000:14 — Insert:207
444. NSpacer .375 OD x .250:4 — Insert:222, Insert:223
445. TWasher .375 OD x .03125:15 — Insert:223
446. TWasher .500 OD x .04000:16 — Insert:226
447. NSpacer Black .500 OD x .125:10 — Insert:257
448. TWasher .375 OD x .06250:17 — Insert:257
449. NSpacer Black .500 OD x .125:11 — Insert:259, Insert:316
450. TWasher .375 OD x .06250:18 — Insert:259
451. NSpacer Black .500 OD x .125:12 — Insert:264, Insert:314
452. NSpacer Black .500 OD x .125:13 — Insert:269
453. Nut Nylock:145 — Insert:442
454. Nut Nylock:146 — Insert:443
455. Nut Nylock:147
456. Nut Nylock:148 — Insert:444
457. Nut Nylock:150
458. Nut Nylock:151 — Insert:446
459. Nut Nylock:152 — Insert:445
460. Nut Nylock:153 — Insert:447
461. Nut Nylock:97 — Insert:338
462. Nut Nylock:98 — Insert:337
463. Nut Nylock:99 — Insert:339
464. Nut Thin Nylock:13 — Insert:174
465. Nut Thin Nylock:14 — Insert:175
466. Nut Thin Nylock:15 — Insert:184
467. Nut Thin Nylock:16 — Insert:183
468. Nut Nylock:49 — Insert:180, Insert:181
469. Nut Nylock:50 — Insert:182
470. Nut Nylock:51 — Insert:206, Insert:207
471. Nut Thin Nylock:17 — Insert:209
472. Nut Thin Nylock:18 — Insert:215
473. Nut Thin Nylock:19 — Insert:216
474. Nut Thin Nylock:20 — Insert:217
475. Nut Thin Nylock:21 — Insert:218
476. Nut Thin Nylock:22 — Insert:219
477. Nut Thin Nylock:23 — Insert:220
478. Nut Nylock:52 — Insert:225, Insert:226
479. Nut Nylock:53 — Insert:227
480. Nut Nylock:54 — Insert:228
481. Nut Nylock:55 — Insert:233
482. Nut Nylock:56 — Insert:234
483. Nut Nylock:57 — Insert:235
484. Nut Nylock:58 — Insert:236
485. Nut Nylock:59 — Insert:237
486. Nut Nylock:60 — Insert:238
487. Nut Nylock:61 — Insert:239
488. Nut Nylock:62 — Insert:240
489. Nut Nylock:63 — Insert:241
490. Nut Nylock:64 — Insert:248
491. Nut Nylock:65 — Insert:249
492. Nut Nylock:66 — Insert:250
493. Nut Nylock:67 — Insert:251
494. Nut Nylock:68 — Insert:252
495. Nut Nylock:69 — Insert:253
496. Nut Nylock:70 — Insert:254
497. Nut Nylock:71 — Insert:255
498. Nut Nylock:72 — Insert:256
499. Nut Nylock:73
500. Nut Nylock:74 — Insert:270
501. Nut Nylock:75 — Insert:271
502. Nut Nylock:76 — Insert:272
503. Nut Nylock:77 — Insert:273
504. Nut Nylock:78
505. Nut Nylock:79
506. Nut Nylock:80
507. Nut Nylock:81 — Insert:282
508. Nut Nylock:82 — Insert:283
509. Nut Nylock:83 — Insert:284
510. Nut Nylock:84 — Insert:285
511. Nut Nylock:85 — Insert:286
512. Nut Nylock:86 — Insert:287
513. Nut Nylock:87 — Insert:288
514. Nut Nylock:88 — Insert:289
515. Nut Nylock:89 — Insert:292
516. Nut Nylock:90 — Insert:293
517. Nut Nylock:91 — Insert:294
518. Nut Nylock:92 — Insert:295
519. Nut Nylock:93 — Insert:296
520. Nut Nylock:94 — Insert:297
521. Nut Nylock:95 — Insert:298
522. Nut Nylock:96 — Insert:299
523. SScrew Star Smooth 1.750:100 — Insert:548
524. SScrew Star Smooth 1.750:101 — Insert:549
525. SScrew Star Smooth 1.750:102 — Insert:551
526. SScrew Star Smooth 1.750:103 — Insert:550
527. SScrew Star Smooth 1.500:69 — Insert:336
528. SScrew Star Smooth .250:64 — Insert:319
529. SScrew Star Smooth .250:65 — Insert:317
530. SScrew Star Smooth .250:66 — Insert:318
531. SScrew Star Smooth .250:67 — Insert:320
532. SScrew Star Smooth .875:35 — Insert:274
533. SScrew Star Smooth .875:36 — Insert:275
534. SScrew Star Smooth .875:37 — Insert:276
535. SScrew Star Smooth .875:38 — Insert:277
536. SScrew Star Smooth 1.750:39
537. SScrew Star Smooth 1.750:40 — Insert:280
538. SScrew Star Smooth 1.500:41 — Insert:281
539. SScrew Star Smooth 1.750:42
540. SScrew Star Smooth 1.500:43 — Insert:290
541. SScrew Star Smooth 1.500:44 — Insert:291
542. SScrew Star Smooth .500:45 — Insert:300
543. SScrew Star Smooth 2.000:46 — Insert:173
544. SScrew Star Smooth .500:47 — Insert:189
545. SScrew Star Smooth .500:48 — Insert:190
546. SScrew Star Smooth 1.000:49 — Insert:200
547. SScrew Star Smooth 1.000:50 — Insert:201
548. SScrew Star Smooth 1.000:51 — Insert:202
549. SScrew Star Smooth 1.000:52 — Insert:203
550. SScrew Star Smooth 2.000:53 — Insert:204
551. SScrew Star Smooth 1.000:54 — Insert:210
552. SScrew Star Smooth 2.000:55 — Insert:208
553. SScrew Star Smooth 1.000:56 — Insert:211
554. SScrew Star Smooth 1.500:57 — Insert:230
555. SScrew Star Smooth 1.500:58 — Insert:231
556. SScrew Star Smooth 1.500:59 — Insert:232
557. SScrew Star Smooth 1.500:60 — Insert:245
558. SScrew Star Smooth 1.500:61 — Insert:246
559. SScrew Star Smooth 1.500:62 — Insert:247
560. SScrew Star Smooth .500:63 — Insert:301
561. Shaft LS 3.5:10 — Insert:329
562. Shaft LS 3.5:6 — Insert:302
563. Shaft LS 3.5:7 — Insert:303
564. Shaft LS 3.5:8 — Insert:304
565. Insert Circle:8 — Insert:179, Insert:180
566. Insert Square:9 — Insert:191, Insert:192
567. Insert Circle:9 — Insert:205, Insert:206
568. Insert Square:10 — Insert:221, Insert:222
569. Insert Circle:10 — Insert:224, Insert:225
570. Insert Square:11 — Insert:262, Insert:264
571. Insert Square:12 — Insert:263, Insert:269
572. Insert Square:13 — Insert:309, Insert:312
573. Insert Square:14 — Insert:310, Insert:313
574. Insert Square:15 — Insert:311
575. Insert Square:16 — Insert:315, Insert:316
## Relationships (660: Insert 596, Flush 24, Mate 17, Angle 13, RelateRotation 6, Tangent 4)
- Insert:1: Alu C 1x3x1x29:1 ↔ Alu C 1x2x1x27:2
- Insert:10: Alu C 1x2x1x27:2 ↔ SScrew Star Smooth 2.000:1
- Insert:11: Alu C 1x2x1x27:2 ↔ Nut Thin Nylock:1
- Insert:12: DriveGear1:1 ↔ Insert Circle:1
- Insert:13: Insert Circle:1 ↔ Nut Thin Nylock:1
- Angle:1 (-90 deg): Alu C 1x3x1x29:1 ↔ Alu C 1x2x1x27:2
- Insert:17: Alu C 1x2x1x27:2 ↔ Nut Thin Nylock:3
- Insert:18: DriveGear1:2 ↔ Insert Circle:3
- Insert:19: Insert Circle:3 ↔ Nut Thin Nylock:3
- Insert:20: DriveGear1:1 ↔ 2.75 Omni AS, No Insert:1
- Insert:21: DriveGear2:1 ↔ Insert Square:1
- Insert:22: NSpacer Black .500 OD x .125:1 ↔ Insert Square:1
- Insert:23: NSpacer Black .500 OD x .125:1 ↔ TWasher .375 OD x .06250:1
- Insert:24: Alu C 1x2x1x27:2 ↔ TWasher .375 OD x .06250:1
- Insert:25: DriveGear2:1 ↔ SScrew Star Smooth .250:2
- Insert:26: 2.75 Omni AS, No Insert:1 ↔ Insert Circle:4
- Insert:29: Alu C 1x3x1x29:1 ↔ Alu C 1x2x1x29:3
- Insert:30: Insert Circle:4 ↔ Nut Nylock:1
- Insert:31: TWasher .500 OD x .04000:2 ↔ Nut Nylock:1
- Insert:32: Alu C 1x2x1x29:3 ↔ Nut Nylock:2
- Insert:33: Alu C 1x2x1x29:3 ↔ Bearing Flat:1
- Insert:34: Alu C 1x2x1x29:3 ↔ Bearing Flat:1
- Insert:35: Alu C 1x2x1x29:3 ↔ SScrew Star Smooth .500:4
- Insert:36: Alu C 1x2x1x29:3 ↔ SScrew Star Smooth .500:3
- Insert:37: Bearing Flat:1 ↔ Nut Thin Nylock:4
- Insert:38: Bearing Flat:1 ↔ Nut Thin Nylock:5
- Insert:39: DriveGear2:1 ↔ Insert Square:2
- Insert:40: NSpacer .375 OD x .250:1 ↔ Insert Square:2
- Insert:41: NSpacer .375 OD x .250:1 ↔ TWasher .375 OD x .03125:3
- Insert:44: TWasher .375 OD x .06250:4 ↔ NSpacer Black .500 OD x .125:2
- Insert:45: Alu C 1x2x1x27:2 ↔ TWasher .375 OD x .06250:4
- Insert:46: DriveGear2:2 ↔ Insert Square:3
- Insert:47: NSpacer Black .500 OD x .125:2 ↔ Insert Square:3
- Insert:48: Alu C 1x2x1x29:3 ↔ Bearing Flat:2
- Insert:49: Alu C 1x2x1x29:3 ↔ Bearing Flat:2
- Insert:50: DriveGear1:2 ↔ 2.75 Omni AS, No Insert:2
- Insert:51: DriveGear1:2 ↔ 2.75 Omni AS, No Insert:2
- Insert:52: DriveGear1:2 ↔ 2.75 Omni AS, No Insert:2
- Insert:54: DriveGear1:2 ↔ 2.75 Omni AS, No Insert:2
- Insert:55: DriveGear1:2 ↔ SScrew Star Smooth 1.000:5
- Insert:56: DriveGear1:2 ↔ SScrew Star Smooth 1.000:6
- Insert:57: DriveGear1:1 ↔ SScrew Star Smooth 1.000:8
- Insert:58: DriveGear1:1 ↔ SScrew Star Smooth 1.000:7
- Insert:59: Alu C 1x2x1x27:2 ↔ SScrew Star Smooth 2.000:9
- Insert:60: 2.75 Omni AS, No Insert:2 ↔ Insert Circle:5
- Insert:61: Insert Circle:5 ↔ Nut Nylock:3
- Insert:62: TWasher .500 OD x .04000:5 ↔ Nut Nylock:3
- Insert:63: Alu C 1x2x1x27:2 ↔ SScrew Star Smooth 2.000:10
- Insert:64: Alu C 1x2x1x27:2 ↔ Nut Thin Nylock:6
- Insert:65: DriveGear1:3 ↔ Insert Circle:6
- Insert:66: DriveGear1:3 ↔ SScrew Star Smooth 1.000:13
- Insert:67: DriveGear1:3 ↔ SScrew Star Smooth 1.000:12
- Insert:68: Insert Circle:6 ↔ Nut Thin Nylock:6
- Insert:69: DriveGear1:3 ↔ 2.75 Omni AS, No Insert:3
- Insert:70: DriveGear1:3 ↔ 2.75 Omni AS, No Insert:3
- Insert:71: DriveGear1:3 ↔ 2.75 Omni AS, No Insert:3
- Insert:72: 2.75 Omni AS, No Insert:1 ↔ Nut Thin Nylock:7
- Insert:73: 2.75 Omni AS, No Insert:1 ↔ Nut Thin Nylock:8
- Insert:74: 2.75 Omni AS, No Insert:2 ↔ Nut Thin Nylock:9
- Insert:75: 2.75 Omni AS, No Insert:2 ↔ Nut Thin Nylock:10
- Insert:76: 2.75 Omni AS, No Insert:3 ↔ Nut Thin Nylock:11
- Insert:77: 2.75 Omni AS, No Insert:3 ↔ Nut Thin Nylock:12
- Insert:78: DriveGear2:2 ↔ Insert Square:4
- Insert:79: NSpacer .375 OD x .250:2 ↔ Insert Square:4
- Insert:80: NSpacer .375 OD x .250:2 ↔ TWasher .375 OD x .03125:6
- Insert:81: DriveGear2:2 ↔ SScrew Star Smooth .250:14
- Insert:82: 2.75 Omni AS, No Insert:3 ↔ Insert Circle:7
- Insert:83: Insert Circle:7 ↔ Nut Nylock:4
- Insert:84: TWasher .500 OD x .04000:7 ↔ Nut Nylock:4
- Insert:85: Alu C 1x2x1x29:3 ↔ Nut Nylock:6
- Insert:86: Alu C 1x2x1x29:3 ↔ Nut Nylock:5
- Insert:87: Alu C 1x2x1x27:2 ↔ CapOriginal:1
- Mate:1: Alu C 1x2x1x27:2 ↔ CapOriginal:1
- Angle:2 (180 deg): Alu C 1x2x1x27:2 ↔ CapOriginal:1
- Insert:88: CapOriginal:1 ↔ SScrew Star Smooth 1.500:15
- Insert:89: CapOriginal:1 ↔ SScrew Star Smooth 1.500:16
- Insert:90: CapOriginal:1 ↔ SScrew Star Smooth 1.500:17
- Insert:91: Alu C 1x2x1x27:2 ↔ Nut Nylock:8
- Insert:92: Alu C 1x2x1x27:2 ↔ Nut Nylock:9
- Insert:93: Alu C 1x2x1x27:2 ↔ Nut Nylock:7
- Insert:94: Alu C 1x2x1x27:2 ↔ Nut Nylock:11
- Insert:95: Alu C 1x2x1x27:2 ↔ Nut Nylock:12
- Insert:96: Alu C 1x2x1x27:2 ↔ Nut Nylock:15
- Insert:97: CapOriginal:1 ↔ Nut Nylock:10
- Insert:98: CapOriginal:1 ↔ Nut Nylock:13
- Insert:99: CapOriginal:1 ↔ Nut Nylock:14
- Insert:101: Alu C 1x2x1x27:2 ↔ CapOriginal:2
- Insert:102: Alu C 1x2x1x27:2 ↔ CapOriginal:2
- Insert:103: CapOriginal:2 ↔ SScrew Star Smooth 1.500:18
- Insert:104: CapOriginal:2 ↔ SScrew Star Smooth 1.500:19
- Insert:105: CapOriginal:2 ↔ SScrew Star Smooth 1.500:20
- Insert:106: CapOriginal:2 ↔ Nut Nylock:16
- Insert:107: CapOriginal:2 ↔ Nut Nylock:17
- Insert:108: CapOriginal:2 ↔ Nut Nylock:18
- Insert:109: Alu C 1x2x1x27:2 ↔ Nut Nylock:19
- Insert:110: Alu C 1x2x1x27:2 ↔ Nut Nylock:20
- Insert:111: Alu C 1x2x1x27:2 ↔ Nut Nylock:21
- Insert:112: Alu C 1x2x1x27:2 ↔ Nut Nylock:22
- Insert:113: Alu C 1x2x1x27:2 ↔ Nut Nylock:23
- Insert:114: Alu C 1x2x1x27:2 ↔ Nut Nylock:24
- Tangent:1 (34.29 mm): DriveGear2:1 ↔ DriveGear2:3
- Flush:1: DriveGear2:1 ↔ DriveGear2:3
- Flush:2: Alu C 1x2x1x29:3 ↔ 3rdAnd4thGearMount:1
- Flush:3: Alu C 1x2x1x29:3 ↔ 3rdAnd4thGearMount:1
- Flush:4: Alu C 1x2x1x29:3 ↔ 3rdAnd4thGearMount:1
- Insert:115: DriveGear2:3 ↔ Insert Square:5
- Insert:116: NSpacer Black .500 OD x .125:3 ↔ Insert Square:5
- Insert:117: NSpacer Black .500 OD x .125:3 ↔ TWasher .375 OD x .06250:8
- Tangent:2 (34.29 mm): DriveGear2:3 ↔ DriveGear2:4
- Flush:6: DriveGear2:3 ↔ DriveGear2:4
- Insert:119: 3rdAnd4thGearMount:1 ↔ DriveGear2:4
- Insert:120: DriveGear2:4 ↔ Insert Square:6
- Insert:121: NSpacer Black .500 OD x .125:4 ↔ Insert Square:6
- Insert:122: NSpacer Black .500 OD x .125:4 ↔ TWasher .375 OD x .06250:9
- Insert:123: Alu C 1x2x1x27:2 ↔ CombinedMotorMount:1
- Insert:124: Alu C 1x2x1x27:2 ↔ CombinedMotorMount:1
- Insert:125: DriveGear2:3 ↔ Insert Square:7
- Insert:126: DriveGear2:4 ↔ Insert Square:8
- Insert:127: 3rdAnd4thGearMount:1 ↔ Bearing Flat:3
- Insert:128: 3rdAnd4thGearMount:1 ↔ Bearing Flat:3
- Insert:129: 3rdAnd4thGearMount:1 ↔ Bearing Flat:4
- Insert:130: 3rdAnd4thGearMount:1 ↔ Bearing Flat:4
- Insert:131: NSpacer Black .500 OD x .125:6 ↔ Insert Square:7
- Insert:132: NSpacer Black .500 OD x .125:7 ↔ Insert Square:8
- Insert:133: Bearing Flat:4 ↔ Nut Nylock:26
- Insert:134: Bearing Flat:4 ↔ Nut Nylock:27
- Insert:135: Bearing Flat:3 ↔ Nut Nylock:28
- Insert:136: Bearing Flat:3 ↔ Nut Nylock:29
- Insert:137: 3rdAnd4thGearMount:1 ↔ SScrew Star Smooth .875:21
- Insert:138: 3rdAnd4thGearMount:1 ↔ SScrew Star Smooth .875:22
- Insert:139: 3rdAnd4thGearMount:1 ↔ SScrew Star Smooth .875:23
- Insert:140: 3rdAnd4thGearMount:1 ↔ SScrew Star Smooth .875:24
- Insert:141: Alu C 1x3x1x29:1 ↔ Nut Nylock:30
- Insert:144: Alu C 1x3x1x29:1 ↔ SScrew Star Smooth 1.750:25
- Insert:145: Alu C 1x2x1x29:3 ↔ SScrew Star Smooth 1.750:26
- Insert:146: Alu C 1x2x1x29:3 ↔ SScrew Star Smooth 1.500:27
- Insert:147: Alu C 1x2x1x29:3 ↔ Nut Nylock:36
- Insert:148: Alu C 1x2x1x29:3 ↔ Nut Nylock:37
- Insert:149: Alu C 1x2x1x29:3 ↔ Nut Nylock:33
- Insert:150: Alu C 1x2x1x29:3 ↔ Nut Nylock:34
- Insert:151: Alu C 1x2x1x29:3 ↔ Nut Nylock:35
- Insert:152: Alu C 1x2x1x29:3 ↔ Nut Nylock:38
- Insert:153: DriveGear2:4 ↔ SScrew Star Smooth .250:28
- Insert:154: DriveGear2:3 ↔ SScrew Star Smooth .250:29
- Insert:155: Alu C 1x3x1x29:1 ↔ SScrew Star Smooth 1.750:30
- Insert:156: Alu C 1x2x1x27:2 ↔ Nut Nylock:39
- Insert:157: Alu C 1x2x1x27:2 ↔ Nut Nylock:40
- Insert:158: CombinedMotorMount:1 ↔ SScrew Star Smooth 1.500:31
- Insert:159: CombinedMotorMount:1 ↔ SScrew Star Smooth 1.500:32
- Insert:160: Alu C 1x2x1x27:2 ↔ Nut Nylock:41
- Insert:161: Alu C 1x2x1x27:2 ↔ Nut Nylock:42
- Insert:162: Alu C 1x2x1x27:2 ↔ Nut Nylock:43
- Insert:163: Alu C 1x2x1x27:2 ↔ Nut Nylock:44
- Insert:164: Alu C 1x2x1x27:2 ↔ Nut Nylock:46
- Insert:165: Alu Angle 1x1x21:2 ↔ Nut Nylock:45
- Insert:166: Bearing Flat:2 ↔ Nut Nylock:47
- Insert:167: Bearing Flat:2 ↔ Nut Nylock:48
- Insert:168: Alu C 1x2x1x29:3 ↔ SScrew Star Smooth .500:33
- Insert:169: Alu C 1x2x1x29:3 ↔ SScrew Star Smooth .500:34
- Insert:170: 3rdAnd4thGearMount:1 ↔ Shaft LS 3.5:2
- Insert:171: 3rdAnd4thGearMount:1 ↔ Shaft LS 3.5:4
- Insert:172: Bearing Flat:1 ↔ Shaft LS 3.5:3
- Insert:173: Alu C 1x2x1x27:1 ↔ SScrew Star Smooth 2.000:46
- Insert:174: Alu C 1x2x1x27:1 ↔ Nut Thin Nylock:13
- Insert:175: Alu C 1x2x1x27:1 ↔ Nut Thin Nylock:14
- Insert:176: DriveGear1:4 ↔ 2.75 Omni AS, No Insert:4
- Insert:177: Alu C 1x2x1x27:1 ↔ TWasher .375 OD x .06250:10
- Insert:178: NSpacer Black .500 OD x .125:8 ↔ TWasher .375 OD x .06250:10
- Insert:179: 2.75 Omni AS, No Insert:4 ↔ Insert Circle:8
- Insert:180: Nut Nylock:49 ↔ Insert Circle:8
- Insert:181: TWasher .500 OD x .04000:11 ↔ Nut Nylock:49
- Insert:182: Alu C 1x2x1x29:5 ↔ Nut Nylock:50
- Insert:183: Bearing Flat:5 ↔ Nut Thin Nylock:16
- Insert:184: Bearing Flat:5 ↔ Nut Thin Nylock:15
- Insert:185: Alu C 1x2x1x29:5 ↔ Bearing Flat:5
- Insert:186: Alu C 1x2x1x29:5 ↔ Bearing Flat:5
- Insert:187: Alu C 1x2x1x29:5 ↔ Bearing Flat:6
- Insert:188: Alu C 1x2x1x29:5 ↔ Bearing Flat:6
- Insert:189: Alu C 1x2x1x29:5 ↔ SScrew Star Smooth .500:47
- Insert:190: Alu C 1x2x1x29:5 ↔ SScrew Star Smooth .500:48
- Insert:191: DriveGear2:5 ↔ Insert Square:9
- Insert:192: NSpacer .375 OD x .250:3 ↔ Insert Square:9
- Insert:193: NSpacer .375 OD x .250:3 ↔ TWasher .375 OD x .03125:12
- Insert:194: Alu C 1x2x1x27:1 ↔ TWasher .375 OD x .06250:13
- Insert:195: TWasher .375 OD x .06250:13 ↔ NSpacer Black .500 OD x .125:9
- Insert:196: DriveGear1:5 ↔ 2.75 Omni AS, No Insert:5
- Insert:197: DriveGear1:5 ↔ 2.75 Omni AS, No Insert:5
- Insert:198: DriveGear1:5 ↔ 2.75 Omni AS, No Insert:5
- Insert:199: DriveGear1:5 ↔ 2.75 Omni AS, No Insert:5
- Insert:200: DriveGear1:5 ↔ SScrew Star Smooth 1.000:49
- Insert:201: DriveGear1:5 ↔ SScrew Star Smooth 1.000:50
- Insert:202: DriveGear1:4 ↔ SScrew Star Smooth 1.000:51
- Insert:203: DriveGear1:4 ↔ SScrew Star Smooth 1.000:52
- Insert:204: Alu C 1x2x1x27:1 ↔ SScrew Star Smooth 2.000:53
- Insert:205: 2.75 Omni AS, No Insert:5 ↔ Insert Circle:9
- Insert:206: Nut Nylock:51 ↔ Insert Circle:9
- Insert:207: TWasher .500 OD x .04000:14 ↔ Nut Nylock:51
- Insert:208: Alu C 1x2x1x27:1 ↔ SScrew Star Smooth 2.000:55
- Insert:209: Alu C 1x2x1x27:1 ↔ Nut Thin Nylock:17
- Insert:210: DriveGear1:6 ↔ SScrew Star Smooth 1.000:54
- Insert:211: DriveGear1:6 ↔ SScrew Star Smooth 1.000:56
- Insert:212: DriveGear1:6 ↔ 2.75 Omni AS, No Insert:6
- Insert:213: DriveGear1:6 ↔ 2.75 Omni AS, No Insert:6
- Insert:214: DriveGear1:6 ↔ 2.75 Omni AS, No Insert:6
- Insert:215: 2.75 Omni AS, No Insert:4 ↔ Nut Thin Nylock:18
- Insert:216: 2.75 Omni AS, No Insert:4 ↔ Nut Thin Nylock:19
- Insert:217: 2.75 Omni AS, No Insert:5 ↔ Nut Thin Nylock:20
- Insert:218: 2.75 Omni AS, No Insert:5 ↔ Nut Thin Nylock:21
- Insert:219: 2.75 Omni AS, No Insert:6 ↔ Nut Thin Nylock:22
- Insert:220: 2.75 Omni AS, No Insert:6 ↔ Nut Thin Nylock:23
- Insert:221: DriveGear2:6 ↔ Insert Square:10
- Insert:222: NSpacer .375 OD x .250:4 ↔ Insert Square:10
- Insert:223: NSpacer .375 OD x .250:4 ↔ TWasher .375 OD x .03125:15
- Insert:224: 2.75 Omni AS, No Insert:6 ↔ Insert Circle:10
- Insert:225: Nut Nylock:52 ↔ Insert Circle:10
- Insert:226: TWasher .500 OD x .04000:16 ↔ Nut Nylock:52
- Insert:227: Alu C 1x2x1x29:5 ↔ Nut Nylock:53
- Insert:228: Alu C 1x2x1x29:5 ↔ Nut Nylock:54
- Insert:229: Alu C 1x2x1x27:1 ↔ CapOriginal:3
- Angle:3 (180 deg): Alu C 1x2x1x27:1 ↔ CapOriginal:3
- Insert:230: CapOriginal:3 ↔ SScrew Star Smooth 1.500:57
- Insert:231: CapOriginal:3 ↔ SScrew Star Smooth 1.500:58
- Insert:232: CapOriginal:3 ↔ SScrew Star Smooth 1.500:59